# Autodesk Inventor assembly: assembled
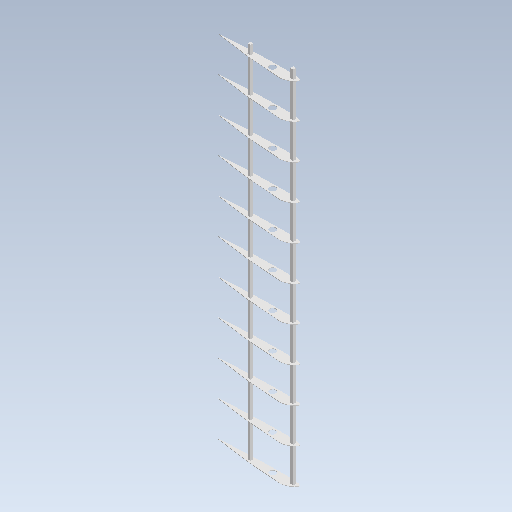
[picture p0: Inventor's stored thumbnail of the model, 512x512]
Saved by Autodesk Inventor 2021 (Build 250183000, 183)
## iProperties
Created: 2021-03-06
Part Number: assembled
Document SubType Name: Assembly
Designer: Ferdinand Hubbard
Author: Ferdinand Hubbard
## Documents named in this file (3)
- C:\Users\Ferdinand Hubbard\Desktop\solarplane\cad\right wing\right wing long.iam
- C:\Users\Ferdinand Hubbard\Desktop\solarplane\cad\airfoil.ipt
- C:\Users\Ferdinand Hubbard\Desktop\solarplane\cad\side long wood spar.ipt
## Components (13 placed, 2 different names)
1. side long wood spar:1 — Mate:2, Mate:4, Mate:7, Mate:10, Mate:13, Mate:16, Mate:18, Mate:21, Mate:24, Mate:27, Mate:30, Mate:33
2. side long wood spar:2 — Mate:1, Mate:3, Mate:6, Mate:9, Mate:12, Mate:15, Mate:17, Mate:20, Mate:23, Mate:26, Mate:29, Mate:32
3. airfoil:1 — Mate:1, Mate:2, Mate:3, Mate:4, Mate:5
4. airfoil:2 — Mate:5, Mate:6, Mate:7, Mate:8
5. airfoil:3 — Mate:8, Mate:9, Mate:10, Mate:11
6. airfoil:4 — Mate:11, Mate:12, Mate:13, Mate:14
7. airfoil:5 — Mate:14, Mate:15, Mate:16, Mate:19
8. airfoil:6 — Mate:17, Mate:18, Mate:19, Mate:22
9. airfoil:7 — Mate:20, Mate:21, Mate:22, Mate:25
10. airfoil:8 — Mate:23, Mate:24, Mate:25, Mate:28
11. airfoil:9 — Mate:26, Mate:27, Mate:28, Mate:31
12. airfoil:10 — Mate:29, Mate:30, Mate:31, Mate:34
13. airfoil:11 — Mate:32, Mate:33, Mate:34
## Relationships (34: Mate 34)
- Mate:1: side long wood spar:2 ↔ airfoil:1
- Mate:2: side long wood spar:1 ↔ airfoil:1
- Mate:3: side long wood spar:2 ↔ airfoil:1
- Mate:4: side long wood spar:1 ↔ airfoil:1
- Mate:5 (156.5 mm): airfoil:1 ↔ airfoil:2
- Mate:6: side long wood spar:2 ↔ airfoil:2
- Mate:7: side long wood spar:1 ↔ airfoil:2
- Mate:8 (156.5 mm): airfoil:2 ↔ airfoil:3
- Mate:9: side long wood spar:2 ↔ airfoil:3
- Mate:10: side long wood spar:1 ↔ airfoil:3
- Mate:11 (156.5 mm): airfoil:3 ↔ airfoil:4
- Mate:12: side long wood spar:2 ↔ airfoil:4
- Mate:13: side long wood spar:1 ↔ airfoil:4
- Mate:14 (156.5 mm): airfoil:4 ↔ airfoil:5
- Mate:15: side long wood spar:2 ↔ airfoil:5
- Mate:16: side long wood spar:1 ↔ airfoil:5
- Mate:17: side long wood spar:2 ↔ airfoil:6
- Mate:18: side long wood spar:1 ↔ airfoil:6
- Mate:19 (156.5 mm): airfoil:5 ↔ airfoil:6
- Mate:20: side long wood spar:2 ↔ airfoil:7
- Mate:21: side long wood spar:1 ↔ airfoil:7
- Mate:22 (156.5 mm): airfoil:6 ↔ airfoil:7
- Mate:23: side long wood spar:2 ↔ airfoil:8
- Mate:24: side long wood spar:1 ↔ airfoil:8
- Mate:25 (156.5 mm): airfoil:7 ↔ airfoil:8
- Mate:26: side long wood spar:2 ↔ airfoil:9
- Mate:27: side long wood spar:1 ↔ airfoil:9
- Mate:28 (156.5 mm): airfoil:8 ↔ airfoil:9
- Mate:29: side long wood spar:2 ↔ airfoil:10
- Mate:30: side long wood spar:1 ↔ airfoil:10
- Mate:31 (156.5 mm): airfoil:9 ↔ airfoil:10
- Mate:32: side long wood spar:2 ↔ airfoil:11
- Mate:33: side long wood spar:1 ↔ airfoil:11
- Mate:34 (156.5 mm): airfoil:10 ↔ airfoil:11
